# Autodesk Inventor assembly: 2016_IEEE_SouteastCon_Court final_left
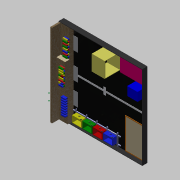
[picture p0: Inventor's stored thumbnail of the model, 180x180]
Saved by Autodesk Inventor 2015 (Build 190159000, 159)
## iProperties
Created: 2015-03-03
Part Number: 2016_IEEE_SouteastCon_Court final_left
Document SubType Name: Assembly
Designer: Vukica
Author: Vukica
## Documents named in this file (15)
- D:\Dropbox\Dropbox\Service\IEEE\!Final Rules\2016Hardware_Court_v8-aug12\2016_IEEE_SouteastCon_Court final_left.iam
- D:\Dropbox\Dropbox\Service\IEEE\!Final Rules\2016Hardware_Court_v8-aug12\Base.ipt
- D:\Dropbox\Dropbox\Service\IEEE\!Final Rules\2016Hardware_Court_v8-aug12\Ship area.ipt
- D:\Dropbox\Dropbox\Service\IEEE\!Final Rules\2016Hardware_Court_v8-aug12\Starting position pink.ipt
- D:\Dropbox\Dropbox\Service\IEEE\!Final Rules\2016Hardware_Court_v8-aug12\Side 84 in by 6 in by half inch.ipt
- D:\Dropbox\Dropbox\Service\IEEE\!Final Rules\2016Hardware_Court_v8-aug12\Side 120 in by 6 in by half inch.ipt
- D:\Dropbox\Dropbox\Service\IEEE\!Final Rules\2016Hardware_Court_v8-aug12\Hill.ipt
- D:\Dropbox\Dropbox\Service\IEEE\!Final Rules\2016Hardware_Court_v8-aug12\Blue truck.ipt
- D:\Dropbox\Dropbox\Service\IEEE\!Final Rules\2016Hardware_Court_v8-aug12\Tunnel.ipt
- D:\Dropbox\Dropbox\Service\IEEE\!Final Rules\2016Hardware_Court_v8-aug12\Shipping goods QR subassembly.iam
- D:\Dropbox\Dropbox\Service\IEEE\!Final Rules\2016Hardware_Court_v8-aug12\Shipping goods generic subassembly.iam
- D:\Dropbox\Dropbox\Service\IEEE\!Final Rules\2016Hardware_Court_v8-aug12\Shipping goods colors subassembly.iam
- D:\Dropbox\Dropbox\Service\IEEE\!Final Rules\2016Hardware_Court_v8-aug12\Rail truck area subassembly v2.iam
- D:\Dropbox\Dropbox\Service\IEEE\!Final Rules\2016Hardware_Court_v8-aug12\Navigation stripes.ipt
- D:\Dropbox\Dropbox\Service\IEEE\!Final Rules\2016Hardware_Court_v8-aug12\Dead reckoning line.ipt
## Components (16 placed, 14 different names)
1. Base:1 — Mate:2, Mate:4, Flush:8, Flush:11, Mate:9, Flush:12, Flush:13, Flush:15, Mate:10, Mate:11, Flush:16, Flush:18, Mate:12, Mate:30, Mate:62, Mate:126, Mate:127, Mate:136, Mate:142, Mate:154, Flush:25, Flush:26
2. Ship area:2 — Mate:2, Mate:120, Mate:149
3. Starting position pink:1 — Mate:4, Flush:8, Mate:128, Mate:150, Mate:152
4. Side 84 in by 6 in by half inch:1 — Mate:11, Flush:16, Flush:17, Mate:120, Mate:134
5. Side 84 in by 6 in by half inch:2 — Flush:18, Mate:12, Flush:19, Mate:143
6. Side 120 in by 6 in by half inch:1 — Flush:13, Flush:15, Mate:10, Flush:17, Mate:150, Mate:151, Mate:156
7. Side 120 in by 6 in by half inch:2 — Flush:11, Mate:9, Flush:12, Flush:19, Mate:141, Mate:149, Mate:153
8. Barge:1 — Mate:141, Mate:142, Mate:143, Mate:144, Mate:145, Mate:146, Flush:20, Flush:21, Flush:22, Flush:23, Mate:147, Mate:148, Mate:155
9. Blue truck:2 — Mate:30, Mate:134, Mate:152
10. Tunnel:1 — Mate:62, Mate:126, Mate:127, Mate:128, Mate:151
11. Shipping goods QR subassembly:2 [sub-assembly] — Mate:145, Flush:21
12. Shipping goods generic subassembly:1 [sub-assembly] — Mate:144, Flush:20, Flush:23
13. Shipping goods colors subassembly:1 [sub-assembly] — Mate:146, Flush:22, Mate:148
14. Rail truck area subassembly v2:1 [sub-assembly] — Mate:136, Mate:147, Mate:153
15. Navigation stripes:1 — Mate:154, Mate:155, Mate:156
16. Dead reckoning line:1 — Flush:25, Flush:26
## Relationships (45: Mate 30, Flush 15)
- Mate:2: Base:1 ↔ Ship area:2
- Mate:4: Base:1 ↔ Starting position pink:1
- Flush:8: Base:1 ↔ Starting position pink:1
- Flush:11: Base:1 ↔ Side 120 in by 6 in by half inch:2
- Mate:9: Base:1 ↔ Side 120 in by 6 in by half inch:2
- Flush:12: Base:1 ↔ Side 120 in by 6 in by half inch:2
- Flush:13: Base:1 ↔ Side 120 in by 6 in by half inch:1
- Flush:15: Base:1 ↔ Side 120 in by 6 in by half inch:1
- Mate:10: Base:1 ↔ Side 120 in by 6 in by half inch:1
- Mate:11: Base:1 ↔ Side 84 in by 6 in by half inch:1
- Flush:16: Base:1 ↔ Side 84 in by 6 in by half inch:1
- Flush:17: Side 84 in by 6 in by half inch:1 ↔ Side 120 in by 6 in by half inch:1
- Flush:18: Base:1 ↔ Side 84 in by 6 in by half inch:2
- Mate:12: Base:1 ↔ Side 84 in by 6 in by half inch:2
- Flush:19: Side 84 in by 6 in by half inch:2 ↔ Side 120 in by 6 in by half inch:2
- Mate:30: Base:1 ↔ Blue truck:2
- Mate:62: Base:1 ↔ Tunnel:1
- Mate:120: Ship area:2 ↔ Side 84 in by 6 in by half inch:1
- Mate:126: Base:1 ↔ Tunnel:1
- Mate:127: Base:1 ↔ Tunnel:1
- Mate:128: Starting position pink:1 ↔ Tunnel:1
- Mate:134: Side 84 in by 6 in by half inch:1 ↔ Blue truck:2
- Mate:136: Base:1 ↔ Rail truck area subassembly v2:1
- Mate:141: Side 120 in by 6 in by half inch:2 ↔ Barge:1
- Mate:142: Base:1 ↔ Barge:1
- Mate:143: Side 84 in by 6 in by half inch:2 ↔ Barge:1
- Mate:144: Barge:1 ↔ Shipping goods generic subassembly:1
- Mate:145: Barge:1 ↔ Shipping goods QR subassembly:2
- Mate:146: Barge:1 ↔ Shipping goods colors subassembly:1
- Flush:20: Barge:1 ↔ Shipping goods generic subassembly:1
- Flush:21: Barge:1 ↔ Shipping goods QR subassembly:2
- Flush:22: Barge:1 ↔ Shipping goods colors subassembly:1
- Flush:23 (203.2 mm): Barge:1 ↔ Shipping goods generic subassembly:1
- Mate:147: Barge:1 ↔ Rail truck area subassembly v2:1
- Mate:148 (50.8 mm): Barge:1 ↔ Shipping goods colors subassembly:1
- Mate:149: Ship area:2 ↔ Side 120 in by 6 in by half inch:2
- Mate:150: Starting position pink:1 ↔ Side 120 in by 6 in by half inch:1
- Mate:151: Side 120 in by 6 in by half inch:1 ↔ Tunnel:1
- Mate:152: Starting position pink:1 ↔ Blue truck:2
- Mate:153: Side 120 in by 6 in by half inch:2 ↔ Rail truck area subassembly v2:1
- Mate:154: Base:1 ↔ Navigation stripes:1
- Mate:155: Barge:1 ↔ Navigation stripes:1
- Mate:156 (254 mm): Side 120 in by 6 in by half inch:1 ↔ Navigation stripes:1
- Flush:25: Base:1 ↔ Dead reckoning line:1
- Flush:26: Base:1 ↔ Dead reckoning line:1
